# Autodesk Inventor assembly: Модуль_маркера
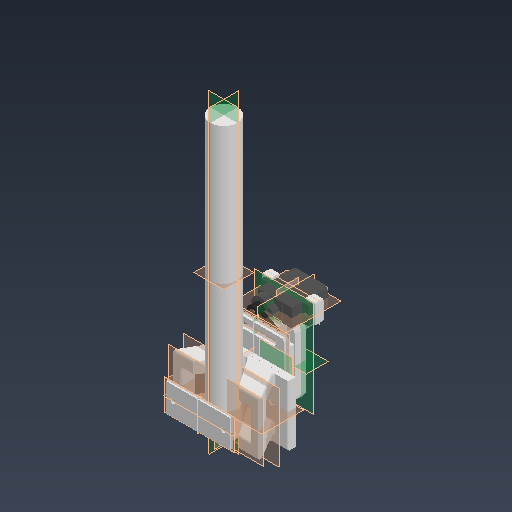
[picture p0: Inventor's stored thumbnail of the model, 512x512]
Saved by Autodesk Inventor 2023.2 (Build 272271030, 271C)
## iProperties
Created: 2026-01-03
Part Number: Модуль_маркера
Document SubType Name: Assembly
Designer: Олег Коноваленко
Author: Олег Коноваленко
## Documents named in this file (10)
- D:\VSOSH_IT_Robotics_ETZ\ETZ\Сonstruction\Модуль_маркера.iam
- D:\VSOSH_IT_Robotics_ETZ\ETZ\Сonstruction\Основание.ipt
- D:\VSOSH_IT_Robotics_ETZ\ETZ\Сonstruction\Направляющая.ipt
- D:\VSOSH_IT_Robotics_ETZ\ETZ\Сonstruction\Каретка.ipt
- D:\VSOSH_IT_Robotics_ETZ\ETZ\Сonstruction\Фанерка_маркера.ipt
- D:\VSOSH_IT_Robotics_ETZ\ETZ\Сonstruction\Крепление_маркера.ipt
- D:\VSOSH_IT_Robotics_ETZ\ETZ\Сonstruction\маркер.ipt
- D:\VSOSH_IT_Robotics_ETZ\ETZ\Сonstruction\DXF\Фиксатор.ipt
- D:\VSOSH_IT_Robotics_ETZ\ETZ\Сonstruction\MG90S Micro Servo Motor.ipt
- D:\VSOSH_IT_Robotics_ETZ\ETZ\Сonstruction\Качалка.ipt
## Components (9 placed, 9 different names)
1. Основание:1 — Совмещение:1, Совмещение:2, Заподлицо:1, Совмещение:3, Совмещение:4, Заподлицо:2, Совмещение:19, Совмещение:20
2. Направляющая:1 — Совмещение:3, Совмещение:4, Заподлицо:2, Совмещение:5, Совмещение:6
3. Каретка:1 — Совмещение:5, Совмещение:6, Совмещение:7, Совмещение:8, Совмещение:9
4. Фанерка_маркера:1 — Совмещение:7, Совмещение:8, Совмещение:9, Совмещение:10, Совмещение:11, Совмещение:12, Совмещение:14, Совмещение:21, Касательность:1
5. Крепление_маркера:1 — Совмещение:10, Совмещение:11, Совмещение:12, Совмещение:13, Совмещение:15, Совмещение:16
6. маркер:1 — Совмещение:13, Совмещение:14
7. Фиксатор:1 — Совмещение:15, Совмещение:16
8. MG90S Micro Servo Motor:1 — Совмещение:17, Совмещение:18, Совмещение:19, Совмещение:20
9. Качалка:1 — Совмещение:17, Совмещение:18, Совмещение:21, Касательность:1
## Relationships (24: Mate 21, Flush 2, Tangent 1)
- Совмещение:1 [Mate]: Основание:1
- Совмещение:2 [Mate]: Основание:1
- Заподлицо:1 [Flush]: Основание:1
- Совмещение:3 [Mate]: Основание:1 ↔ Направляющая:1
- Совмещение:4 [Mate]: Основание:1 ↔ Направляющая:1
- Заподлицо:2 [Flush]: Основание:1 ↔ Направляющая:1
- Совмещение:5 [Mate]: Направляющая:1 ↔ Каретка:1
- Совмещение:6 [Mate]: Направляющая:1 ↔ Каретка:1
- Совмещение:7 [Mate]: Каретка:1 ↔ Фанерка_маркера:1
- Совмещение:8 [Mate]: Каретка:1 ↔ Фанерка_маркера:1
- Совмещение:9 [Mate]: Каретка:1 ↔ Фанерка_маркера:1
- Совмещение:10 [Mate]: Фанерка_маркера:1 ↔ Крепление_маркера:1
- Совмещение:11 [Mate]: Фанерка_маркера:1 ↔ Крепление_маркера:1
- Совмещение:12 [Mate]: Фанерка_маркера:1 ↔ Крепление_маркера:1
- Совмещение:13 [Mate]: Крепление_маркера:1 ↔ маркер:1
- Совмещение:14 [Mate] (19.8 mm): Фанерка_маркера:1 ↔ маркер:1
- Совмещение:15 [Mate]: Крепление_маркера:1 ↔ Фиксатор:1
- Совмещение:16 [Mate]: Крепление_маркера:1 ↔ Фиксатор:1
- Совмещение:17 [Mate]: MG90S Micro Servo Motor:1 ↔ Качалка:1
- Совмещение:18 [Mate]: MG90S Micro Servo Motor:1 ↔ Качалка:1
- Совмещение:19 [Mate]: Основание:1 ↔ MG90S Micro Servo Motor:1
- Совмещение:20 [Mate]: Основание:1 ↔ MG90S Micro Servo Motor:1
- Совмещение:21 [Mate] (1 mm): Фанерка_маркера:1 ↔ Качалка:1
- Касательность:1 [Tangent] (1.5 mm): Фанерка_маркера:1 ↔ Качалка:1
